# Autodesk Inventor assembly: Assembly
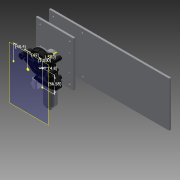
[picture p0: Inventor's stored thumbnail of the model, 180x180]
Saved by Autodesk Inventor 2014 SP1 (Build 180222100, 222)
## iProperties
Created: 2014-02-07
Part Number: Assembly
Document SubType Name: Assembly
Designer: Owner
Author: Owner
## Documents named in this file (6)
- C:\Users\Owner\Documents\GitHub\Team2083-2014-CAD\Winebago Concept\Generation 2\Assembly.iam
- C:\Users\Owner\Documents\GitHub\Team2083-2014-CAD\Winebago Concept\Generation 2\big plate.ipt
- C:\Users\Owner\Documents\GitHub\Team2083-2014-CAD\Winebago Concept\Generation 2\small plate.ipt
- C:\Users\Owner\Documents\GitHub\Team2083-2014-CAD\Winebago Concept\Window Motor\ND Motor Right.ipt
- C:\Users\Owner\Documents\GitHub\Team2083-2014-CAD\Winebago Concept\Generation 2\motor connector.ipt
- C:\Users\Owner\Documents\GitHub\Team2083-2014-CAD\Winebago Concept\3 in bar.ipt
## Components (5 placed, 5 different names)
1. big plate:1 — Mate:1, Mate:2, Mate:3, Mate:4
2. small plate:1 — Mate:1, Mate:2, Mate:3, Mate:4, Mate:5, Mate:6, Mate:7, Flush:1
3. ND Motor Right:1 — Mate:5, Mate:6, Mate:7, Mate:8, Mate:9
4. motor connector:1 — Mate:8, Mate:9, Flush:1, Insert:1
5. 3 in bar:1 — Insert:1
## Relationships (11: Mate 9, Flush 1, Insert 1)
- Mate:1: big plate:1 ↔ small plate:1
- Mate:2: big plate:1 ↔ small plate:1
- Mate:3: big plate:1 ↔ small plate:1
- Mate:4 (38.1 mm): big plate:1 ↔ small plate:1
- Mate:5: small plate:1 ↔ ND Motor Right:1
- Mate:6: small plate:1 ↔ ND Motor Right:1
- Mate:7: small plate:1 ↔ ND Motor Right:1
- Mate:8: ND Motor Right:1 ↔ motor connector:1
- Mate:9 (2.54 mm): ND Motor Right:1 ↔ motor connector:1
- Flush:1 (-12.7 mm): small plate:1 ↔ motor connector:1
- Insert:1: motor connector:1 ↔ 3 in bar:1
